# Autodesk Inventor assembly: ForeArm_hand
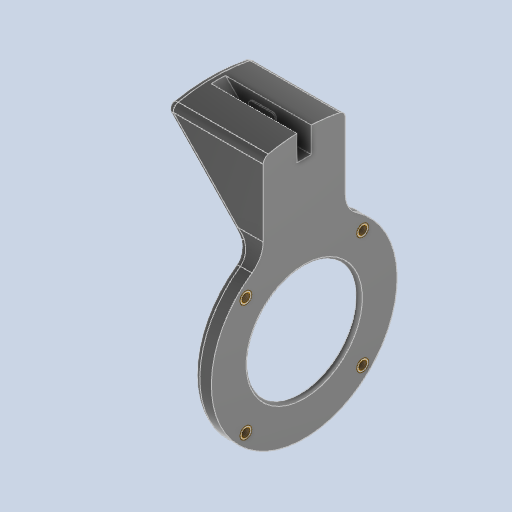
[picture p0: Inventor's stored thumbnail of the model, 512x512]
Saved by Autodesk Inventor 2022.5 (Build 265521000, 521)
## iProperties
Created: 2023-06-02
Part Number: ForeArm_hand
Document SubType Name: Assembly
Designer: Masato Kubotera
Mass: 89.0399 g
Surface Area: 517.759 cm^2
Volume: 65.3623 cm^3
Density: 1.36225 g/cm^3
Author: Masato Kubotera
## Documents named in this file (3)
- C:\Users\Masato\Documents\Inventor\SUSTAINA-OP\ModelingFiles\UpperBody\Arm\ForeArm_hand.iam
- C:\Users\Masato\Documents\Inventor\SUSTAINA-OP\ModelingFiles\COTS\InsertNut\UD-43040.ipt
- C:\Users\Masato\Documents\Inventor\SUSTAINA-OP\ModelingFiles\UpperBody\Arm\ForeArm_hand.ipt
## Components (5 placed, 2 different names)
1. UD-43040:1 — 挿入:1
2. UD-43040:2 — 挿入:2
3. UD-43040:3 — 挿入:3
4. UD-43040:4 — 挿入:4
5. ForeArm_hand:1 — 挿入:1, 挿入:2, 挿入:3, 挿入:4
## Relationships (7: Insert 4, Flush 3)
- [Flush]: ForeArm_hand:1
- [Flush]: ForeArm_hand:1
- [Flush]: ForeArm_hand:1
- 挿入:1 [Insert]: UD-43040:1 ↔ ForeArm_hand:1
- 挿入:2 [Insert]: UD-43040:2 ↔ ForeArm_hand:1
- 挿入:3 [Insert]: UD-43040:3 ↔ ForeArm_hand:1
- 挿入:4 [Insert]: UD-43040:4 ↔ ForeArm_hand:1
